# Autodesk Inventor assembly: Eje-engrane_chico
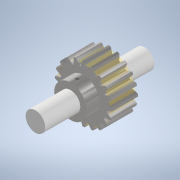
[picture p0: Inventor's stored thumbnail of the model, 180x180]
Saved by Autodesk Inventor 2021 (Build 250183000, 183)
## iProperties
Created: 2021-02-07
Part Number: Eje-engrane_chico
Document SubType Name: Assembly
Designer: rotje
Author: rotje
## Documents named in this file (3)
- C:\Users\rotje\Documents\Inventor\MSF\Eje-engrane_chico.iam
- C:\Users\rotje\Documents\Inventor\MSF\Eje_engrane.ipt
- C:\Users\rotje\Documents\Inventor\MSF\Engranaje recto_20_Dientes.ipt
## Components (2 placed, 2 different names)
1. Eje_engrane:1 — Insertar:1
2. Engranaje recto1:1 — Insertar:1
## Relationships (1: Insert 1)
- Insertar:1 (10 mm): Eje_engrane:1 ↔ Engranaje recto1:1
